# Autodesk Inventor assembly: ròng rọc - Bản 2
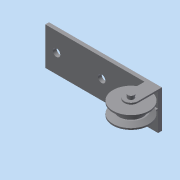
[picture p0: Inventor's stored thumbnail of the model, 180x180]
Saved by Autodesk Inventor 2018 (Build 220112000, 112)
## iProperties
Created: 2020-10-11
Part Number: ròng rọc - Bản 2
Document SubType Name: Assembly
Designer: ASUS
Author: ASUS
## Documents named in this file (3)
- E:\CTU\Skylight\Bản vẽ\Bản vẽ Giếng Trời Tự Động\Bản vẽ 3D\Linh kiện khác\Ròng rọc\ròng rọc - Bản 2.iam
- E:\CTU\Skylight\Bản vẽ\Bản vẽ Giếng Trời Tự Động\Bản vẽ 3D\Linh kiện khác\Ròng rọc\Giá đỡ ròng rọc 2.ipt
- E:\CTU\Skylight\Bản vẽ\Bản vẽ Giếng Trời Tự Động\Bản vẽ 3D\Linh kiện khác\Ròng rọc\Ròng rọc 48mm.ipt
## Components (2 placed, 2 different names)
1. Giá đỡ ròng rọc 2:1 — Mate:1, Mate:2
2. Ròng rọc 48mm:1 — Mate:1, Mate:2
## Relationships (2: Mate 2)
- Mate:1: Giá đỡ ròng rọc 2:1 ↔ Ròng rọc 48mm:1
- Mate:2 (1.5 mm): Giá đỡ ròng rọc 2:1 ↔ Ròng rọc 48mm:1
